# Autodesk Inventor assembly: wheel1_MIR1
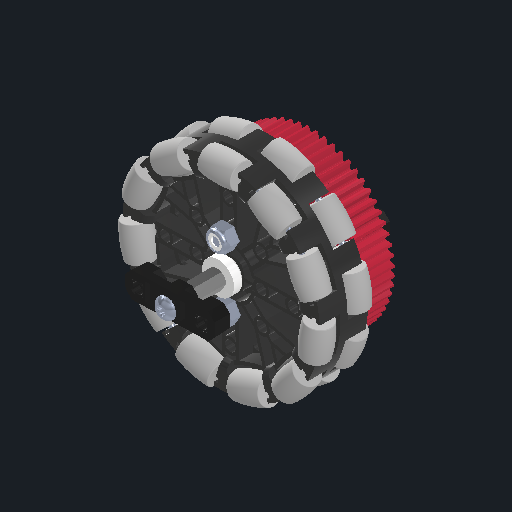
[picture p0: Inventor's stored thumbnail of the model, 512x512]
Saved by Autodesk Inventor 2024 (Build 280153000, 153)
## iProperties
Created: 2023-08-09
Part Number: wheel1_MIR1
Document SubType Name: Assembly
Designer: macbook
Author: macbook
## Documents named in this file (18)
- \\Mac\Home\Desktop\code\7899V-VRC-OVER-UNDER\Cad\VEX-CAD-Inventor-1.4.0\Assembly\v0.2\wheel1_MIR1.iam
- \\Mac\Home\Desktop\code\7899V-VRC-OVER-UNDER\Cad\VEX-CAD-Inventor-1.4.0\Motion\Wheels\Omni Wheel\3.25 Omni AS, Circle_MIR1.iam
- \\Mac\Home\Desktop\code\7899V-VRC-OVER-UNDER\Cad\VEX-CAD-Inventor-1.4.0\Motion\Spacers\Spacer Nylon .500 OD\NSpacer White .500 OD x .250.ipt
- \\Mac\Home\Desktop\code\7899V-VRC-OVER-UNDER\Cad\VEX-CAD-Inventor-1.4.0\Motion\Spacers\Spacer Nylon .500 OD.ipt
- \\Mac\Home\Desktop\code\7899V-VRC-OVER-UNDER\Cad\VEX-CAD-Inventor-1.4.0\Motion\Shaft LS\Bearing Flat_MIR2.ipt
- \\Mac\Home\Desktop\code\7899V-VRC-OVER-UNDER\Cad\VEX-CAD-Inventor-1.4.0\Structure\Hardware\Screw Steel - Star\SScrew Star Smooth .500.ipt
- \\Mac\Home\Desktop\code\7899V-VRC-OVER-UNDER\Cad\VEX-CAD-Inventor-1.4.0\Structure\Hardware\Screw Steel - Star.ipt
- \\Mac\Home\Desktop\code\7899V-VRC-OVER-UNDER\Cad\VEX-CAD-Inventor-1.4.0\Structure\Standoff\Standoff .50.ipt
- \\Mac\Home\Desktop\code\7899V-VRC-OVER-UNDER\Cad\VEX-CAD-Inventor-1.4.0\Structure\Standoff.ipt
- \\Mac\Home\Desktop\code\7899V-VRC-OVER-UNDER\Cad\VEX-CAD-Inventor-1.4.0\Motion\Spacers\Spacer Nylon .313 OD\NSpacer .313 OD x .250.ipt
- \\Mac\Home\Desktop\code\7899V-VRC-OVER-UNDER\Cad\VEX-CAD-Inventor-1.4.0\Motion\Spacers\Spacer Nylon .313 OD.ipt
- \\Mac\Home\Desktop\code\7899V-VRC-OVER-UNDER\Cad\VEX-CAD-Inventor-1.4.0\Motion\Gears\HS Gear\HS 60T Gear, Circle_MIR.iam
- \\Mac\Home\Desktop\code\7899V-VRC-OVER-UNDER\Cad\VEX-CAD-Inventor-1.4.0\Motion\Spacers\Washer Teflon\TWasher .375 OD x .03125.ipt
- \\Mac\Home\Desktop\code\7899V-VRC-OVER-UNDER\Cad\VEX-CAD-Inventor-1.4.0\Motion\Spacers\Washer Teflon.ipt
- \\Mac\Home\Desktop\code\7899V-VRC-OVER-UNDER\Cad\VEX-CAD-Inventor-1.4.0\Structure\Hardware\Screw Steel - Star\SScrew Star Smooth 1.500.ipt
- \\Mac\Home\Desktop\code\7899V-VRC-OVER-UNDER\Cad\VEX-CAD-Inventor-1.4.0\Structure\Hardware\Nut Nylock_MIR2.ipt
- \\Mac\Home\Desktop\code\7899V-VRC-OVER-UNDER\Cad\VEX-CAD-Inventor-1.4.0\Structure\Hardware\Screw Steel - Star\SScrew Star Smooth 2.250.ipt
- \\Mac\Home\Desktop\code\7899V-VRC-OVER-UNDER\Cad\VEX-CAD-Inventor-1.4.0\Motion\Spacers\Spacer Nylon .500 OD\NSpacer White .500 OD x .125.ipt
## Components (18 placed, 12 different names)
1. 3.25 Omni AS, Circle_MIR1:1 [sub-assembly] — Insert:48, Insert:55, Insert:56, Insert:59
2. NSpacer White .500 OD x .250:1 — Insert:36
3. Bearing Flat_MIR2:1 — Insert:47, Insert:46, Insert:36, Insert:58
4. Bearing Flat_MIR2:2 — Insert:47, Insert:46, Insert:43, Insert:45
5. SScrew Star Smooth .500:1 — Insert:43
6. Standoff .50:1 — Insert:45, Insert:60
7. NSpacer .313 OD x .250:1 — Insert:48, Insert:49
8. HS 60T Gear, Circle_MIR:1 [sub-assembly] — Insert:49, Insert:50, Insert:51, Insert:54, Insert:57
9. NSpacer White .500 OD x .250:2 — Insert:50, Insert:53
10. NSpacer White .500 OD x .250:3 — Insert:51, Insert:52
11. TWasher .375 OD x .03125:1 — Insert:53
12. TWasher .375 OD x .03125:2 — Insert:52
13. SScrew Star Smooth 1.500:2 — Insert:54
14. Nut Nylock_MIR2:1 — Insert:55
15. Nut Nylock_MIR2:2 — Insert:56
16. SScrew Star Smooth 1.500:3 — Insert:57
17. SScrew Star Smooth 2.250:4 — Insert:58
18. NSpacer White .500 OD x .125:4 — Insert:60, Insert:59
## Relationships (18: Insert 18)
- Insert:47 (57.15 mm): Bearing Flat_MIR2:1 ↔ Bearing Flat_MIR2:2
- Insert:46 (57.15 mm): Bearing Flat_MIR2:1 ↔ Bearing Flat_MIR2:2
- Insert:43 (1.5875 mm): Bearing Flat_MIR2:2 ↔ SScrew Star Smooth .500:1
- Insert:45: Bearing Flat_MIR2:2 ↔ Standoff .50:1
- Insert:48: 3.25 Omni AS, Circle_MIR1:1 ↔ NSpacer .313 OD x .250:1
- Insert:49: NSpacer .313 OD x .250:1 ↔ HS 60T Gear, Circle_MIR:1
- Insert:36 (1.5875 mm): NSpacer White .500 OD x .250:1 ↔ Bearing Flat_MIR2:1
- Insert:50: HS 60T Gear, Circle_MIR:1 ↔ NSpacer White .500 OD x .250:2
- Insert:51: HS 60T Gear, Circle_MIR:1 ↔ NSpacer White .500 OD x .250:3
- Insert:53: NSpacer White .500 OD x .250:2 ↔ TWasher .375 OD x .03125:1
- Insert:52: NSpacer White .500 OD x .250:3 ↔ TWasher .375 OD x .03125:2
- Insert:54: HS 60T Gear, Circle_MIR:1 ↔ SScrew Star Smooth 1.500:2
- Insert:55: 3.25 Omni AS, Circle_MIR1:1 ↔ Nut Nylock_MIR2:1
- Insert:56: 3.25 Omni AS, Circle_MIR1:1 ↔ Nut Nylock_MIR2:2
- Insert:57: HS 60T Gear, Circle_MIR:1 ↔ SScrew Star Smooth 1.500:3
- Insert:58: Bearing Flat_MIR2:1 ↔ SScrew Star Smooth 2.250:4
- Insert:60: Standoff .50:1 ↔ NSpacer White .500 OD x .125:4
- Insert:59: 3.25 Omni AS, Circle_MIR1:1 ↔ NSpacer White .500 OD x .125:4
